# Autodesk Inventor assembly: Assembly1
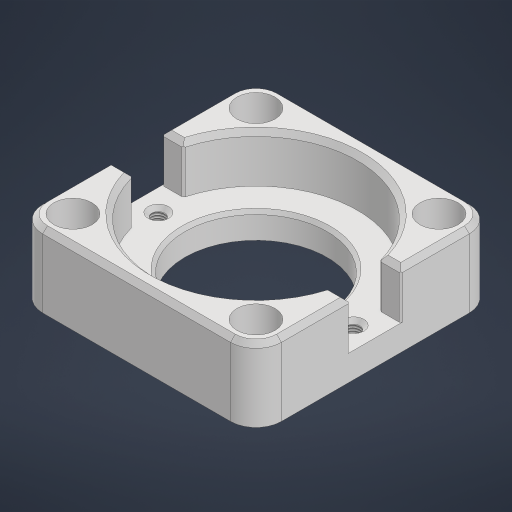
[picture p0: Inventor's stored thumbnail of the model, 512x512]
Saved by Autodesk Inventor 2024.3 (Build 283343000, 343)
## iProperties
Created: 2025-03-15
Part Number: Assembly1
Document SubType Name: Assembly
Designer: fablabadmin
Author: fablabadmin
## Documents named in this file (7)
- C:\Users\fablabadmin\Documents\_Benjamin_S\_3dCAD\HHVerkstad\Temp\Assembly1.iam
- C:\Users\fablabadmin\Documents\_Benjamin_S\_3dCAD\HHVerkstad\Temp\TH1-001.ipt
- C:\Users\fablabadmin\Documents\_Benjamin_S\_3dCAD\_Config\KemmlerVise\OP1-KemmlerVise.iam
- C:\Users\fablabadmin\Documents\_Benjamin_S\_3dCAD\_Config\KemmlerVise\OP2-KemmlerVise.iam
- C:\Users\fablabadmin\Documents\Inventor\Content Center Files\R2024\en-US\StandardJaw\JawSTD-Aluminum 6061.ipt
- C:\Users\fablabadmin\Documents\_Benjamin_S\_3dCAD\HHVerkstad\Temp\Stock.ipt
- C:\Users\fablabadmin\Documents\Inventor\Content Center Files\R2024\en-US\PRL_150x3\31-PRL_150x3-Steel, Carbon.ipt
## Components (7 placed, 6 different names)
1. TH1-001:1 — Flush:5
2. OP1-KemmlerVise:1 [sub-assembly] — Mate:1, Mate:2, Flush:1, Mate:3, Flush:6, Mate:9
3. OP2-KemmlerVise:1 [sub-assembly]
4. JawStandard JawSTD-Aluminum 6061:1 — Mate:1, Flush:1, Flush:2, Mate:3, Mate:4, Mate:6, Mate:7
5. JawStandard JawSTD-Aluminum 6061:2 — Mate:2, Flush:2, Mate:5
6. Stock:1 — Flush:3, Flush:4, Flush:5, Mate:4, Mate:5, Mate:8
7. PRL_150x3 31-PRL_150x3-Steel, Carbon:1 — Mate:6, Flush:6, Mate:7, Mate:8
## Relationships (15: Mate 9, Flush 6)
- Mate:1: OP1-KemmlerVise:1 ↔ JawStandard JawSTD-Aluminum 6061:1
- Mate:2: OP1-KemmlerVise:1 ↔ JawStandard JawSTD-Aluminum 6061:2
- Flush:1: OP1-KemmlerVise:1 ↔ JawStandard JawSTD-Aluminum 6061:1
- Flush:2: JawStandard JawSTD-Aluminum 6061:1 ↔ JawStandard JawSTD-Aluminum 6061:2
- Mate:3: OP1-KemmlerVise:1 ↔ JawStandard JawSTD-Aluminum 6061:1
- Flush:3: Stock:1
- Flush:4: Stock:1
- Flush:5 (-0.5 mm): TH1-001:1 ↔ Stock:1
- Mate:4: JawStandard JawSTD-Aluminum 6061:1 ↔ Stock:1
- Mate:5: JawStandard JawSTD-Aluminum 6061:2 ↔ Stock:1
- Mate:6: JawStandard JawSTD-Aluminum 6061:1 ↔ PRL_150x3 31-PRL_150x3-Steel, Carbon:1
- Flush:6: OP1-KemmlerVise:1 ↔ PRL_150x3 31-PRL_150x3-Steel, Carbon:1
- Mate:7: JawStandard JawSTD-Aluminum 6061:1 ↔ PRL_150x3 31-PRL_150x3-Steel, Carbon:1
- Mate:8: Stock:1 ↔ PRL_150x3 31-PRL_150x3-Steel, Carbon:1
- Mate:9: OP1-KemmlerVise:1
